# Autodesk Inventor assembly: Slope_HighEnd
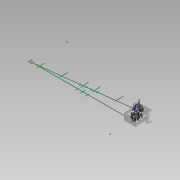
[picture p0: Inventor's stored thumbnail of the model, 180x180]
Saved by Autodesk Inventor 2021 (Build 250183000, 183)
## iProperties
Created: 2021-03-11
Part Number: Slope_HighEnd
Document SubType Name: Assembly
Designer: kumagai
Author: kumagai
## Documents named in this file (4)
- X:\Develop\CAD\PlaRails\SimpleSlope\Slope_HighEnd.iam
- X:\Develop\CAD\PlaRails\SimpleSlope\Slope_HighEnd.ipt
- X:\Develop\CAD\PlaRails\RailJointFemale_filled.ipt
- X:\Develop\CAD\PlaRails\RailJointMale_filled.ipt
## Components (3 placed, 3 different names)
1. Slope_HighEnd:1 — メイト:1, メイト:2, フラッシュ:1, フラッシュ:2, メイト:3, メイト:4
2. RailJointFemale_filled:1 — メイト:1, フラッシュ:1, メイト:3
3. RailJointMale_filled:1 — メイト:2, フラッシュ:2, メイト:4
## Relationships (6: Mate 4, Flush 2)
- メイト:1 [Mate]: Slope_HighEnd:1 ↔ RailJointFemale_filled:1
- メイト:2 [Mate]: Slope_HighEnd:1 ↔ RailJointMale_filled:1
- フラッシュ:1 [Flush]: Slope_HighEnd:1 ↔ RailJointFemale_filled:1
- フラッシュ:2 [Flush]: Slope_HighEnd:1 ↔ RailJointMale_filled:1
- メイト:3 [Mate]: Slope_HighEnd:1 ↔ RailJointFemale_filled:1
- メイト:4 [Mate]: Slope_HighEnd:1 ↔ RailJointMale_filled:1
